# Autodesk Inventor assembly: Full_Model
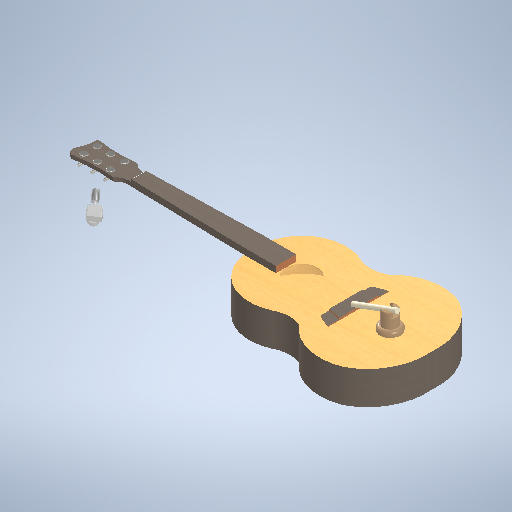
[picture p0: Inventor's stored thumbnail of the model, 512x512]
Saved by Autodesk Inventor 2025.2 (Build 292293000, 293)
## iProperties
Created: 2025-04-14
Part Number: Full_Model
Document SubType Name: Assembly
Designer: 3lin2
Author: 3lin2
## Documents named in this file (6)
- C:\Users\3lin2\OneDrive - University of Illinois - Urbana\Documents\UIUC\ECE 445\Automatic-Guitar-Tuner Github\3D_print\Full_Model.iam
- C:\Users\3lin2\OneDrive - University of Illinois - Urbana\Documents\UIUC\ECE 445\Automatic-Guitar-Tuner Github\3D_print\half_inch_dowel_5inch.ipt
- C:\Users\3lin2\OneDrive - University of Illinois - Urbana\Documents\UIUC\ECE 445\Automatic-Guitar-Tuner Github\3D_print\magnet_mount.ipt
- C:\Users\3lin2\OneDrive - University of Illinois - Urbana\Documents\UIUC\ECE 445\Automatic-Guitar-Tuner Github\3D_print\motor.ipt
- C:\Users\3lin2\OneDrive - University of Illinois - Urbana\Documents\UIUC\ECE 445\Automatic-Guitar-Tuner Github\3D_print\motor-tuningpeg.ipt
- C:\Users\3lin2\OneDrive - University of Illinois - Urbana\Documents\UIUC\ECE 445\Automatic-Guitar-Tuner Github\3D_print\Guitar.ipt
## Components (5 placed, 5 different names)
1. half_inch_dowel_5inch:1 — Angle:1, Mate:2
2. magnet_mount:1 — Angle:1, Mate:1, Mate:2
3. motor:1 — Mate:3, Flush:1, Flush:2
4. motor-tuningpeg:1 — Mate:3, Flush:1, Flush:2
5. Guitar:1 — Mate:1
## Relationships (6: Mate 3, Flush 2, Angle 1)
- Angle:1 (-70 deg): half_inch_dowel_5inch:1 ↔ magnet_mount:1
- Mate:1: magnet_mount:1 ↔ Guitar:1
- Mate:2 (6.985 mm): half_inch_dowel_5inch:1 ↔ magnet_mount:1
- Mate:3 (0.254 mm): motor:1 ↔ motor-tuningpeg:1
- Flush:1: motor:1 ↔ motor-tuningpeg:1
- Flush:2 (7.62 mm): motor:1 ↔ motor-tuningpeg:1
